# Autodesk Inventor assembly: TeflonMagnet
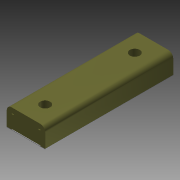
[picture p0: Inventor's stored thumbnail of the model, 180x180]
Saved by Autodesk Inventor 2012 (Build 160160000, 160)
## iProperties
Created: 2012-04-08
Part Number: TeflonMagnet
Document SubType Name: Assembly
Designer: admin
Mass: 40.2234 g
Surface Area: 116.055 cm^2
Volume: 10.928 cm^3
Density: 3.68075 g/cm^3
Author: admin
## Documents named in this file (3)
- C:\Users\admin\Documents\Inventor\SumoJaime2012\TeflonMagnet.iam
- C:\Users\admin\Documents\Inventor\SumoJaime2012\Imported Components\MMR-A-Y8\MMR-A-Y8.ipt
- C:\Users\admin\Documents\Inventor\SumoJaime2012\Teflon01.ipt
## Components (2 placed, 2 different names)
1. MMR-A-Y8:1 — Mate:1, Mate:2, Flush:1, Flush:2
2. Teflon01:1 — Mate:1, Mate:2, Flush:1, Flush:2
## Relationships (4: Mate 2, Flush 2)
- Mate:1: MMR-A-Y8:1 ↔ Teflon01:1
- Mate:2: MMR-A-Y8:1 ↔ Teflon01:1
- Flush:1: MMR-A-Y8:1 ↔ Teflon01:1
- Flush:2: MMR-A-Y8:1 ↔ Teflon01:1
